# Autodesk Inventor assembly: Chessboard Design
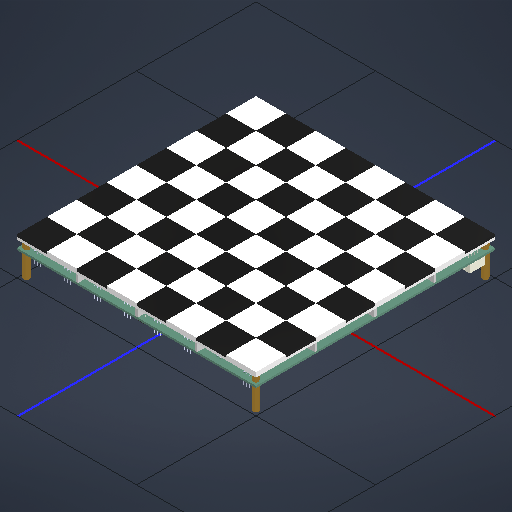
[picture p0: Inventor's stored thumbnail of the model, 512x512]
Saved by Autodesk Inventor 2026 (Build 300175000, 175)
## iProperties
Created: 2025-04-19
Part Number: Chessboard Design
Document SubType Name: Assembly
Designer: ckyiu
Author: ckyiu
## Documents named in this file (6)
- C:\Users\ckyiu\Documents\Projects\Chessboard-Design\Chessboard Design.iam
- C:\Users\ckyiu\Documents\Projects\Chessboard-Design\Assemblies\Chessboard Top.iam
- C:\Users\ckyiu\Documents\Projects\Chessboard-Design\Assemblies\PCBs\Chessboard Hardware Model.iam
- C:\Users\ckyiu\Documents\Projects\Chessboard-Design\Parts\Square Holder Support.ipt
- C:\Users\ckyiu\Documents\Projects\Chessboard-Design\Parts\Standoffs\M2.5 F-F Standoff 6mm.ipt
- C:\Users\ckyiu\Documents\Projects\Chessboard-Design\Parts\Standoffs\M2.5 F-M Standoff 20mm.ipt
## Components (11 placed, 5 different names)
1. Chessboard Top:1 [sub-assembly] — Flush:1, Flush:2, Mate:2
2. Chessboard Hardware Model:1 [sub-assembly] — Flush:1, Flush:2, Flush:3, Flush:4, Mate:1, Insert:1, Angle:1, Insert:2, Angle:2, Insert:3, Angle:3, Insert:4, Angle:4, Insert:5, Insert:6, Insert:7, Insert:8
3. Square Holder Support:1 — Flush:3, Flush:4, Mate:1, Mate:2
4. M2.5 F-F Standoff 6mm:1 — Insert:1, Angle:1, Angle:5
5. M2.5 F-F Standoff 6mm:2 — Insert:4, Angle:4, Angle:7
6. M2.5 F-F Standoff 6mm:3 — Insert:3, Angle:3, Angle:6
7. M2.5 F-F Standoff 6mm:4 — Insert:2, Angle:2, Angle:8
8. M2.5 F-M Standoff 20mm:1 — Insert:5, Angle:5
9. M2.5 F-M Standoff 20mm:2 — Insert:6, Angle:8
10. M2.5 F-M Standoff 20mm:3 — Insert:7, Angle:6
11. M2.5 F-M Standoff 20mm:4 — Insert:8, Angle:7
## Relationships (22: Insert 8, Angle 8, Flush 4, Mate 2)
- Flush:1: Chessboard Top:1 ↔ Chessboard Hardware Model:1
- Flush:2: Chessboard Top:1 ↔ Chessboard Hardware Model:1
- Flush:3: Chessboard Hardware Model:1 ↔ Square Holder Support:1
- Flush:4: Chessboard Hardware Model:1 ↔ Square Holder Support:1
- Mate:1: Chessboard Hardware Model:1 ↔ Square Holder Support:1
- Mate:2: Chessboard Top:1 ↔ Square Holder Support:1
- Insert:1: Chessboard Hardware Model:1 ↔ M2.5 F-F Standoff 6mm:1
- Angle:1 (0 deg): Chessboard Hardware Model:1 ↔ M2.5 F-F Standoff 6mm:1
- Insert:2: Chessboard Hardware Model:1 ↔ M2.5 F-F Standoff 6mm:4
- Angle:2 (0 deg): Chessboard Hardware Model:1 ↔ M2.5 F-F Standoff 6mm:4
- Insert:3: Chessboard Hardware Model:1 ↔ M2.5 F-F Standoff 6mm:3
- Angle:3 (0 deg): Chessboard Hardware Model:1 ↔ M2.5 F-F Standoff 6mm:3
- Insert:4: Chessboard Hardware Model:1 ↔ M2.5 F-F Standoff 6mm:2
- Angle:4 (0 deg): Chessboard Hardware Model:1 ↔ M2.5 F-F Standoff 6mm:2
- Insert:5: Chessboard Hardware Model:1 ↔ M2.5 F-M Standoff 20mm:1
- Insert:6: Chessboard Hardware Model:1 ↔ M2.5 F-M Standoff 20mm:2
- Insert:7: Chessboard Hardware Model:1 ↔ M2.5 F-M Standoff 20mm:3
- Insert:8: Chessboard Hardware Model:1 ↔ M2.5 F-M Standoff 20mm:4
- Angle:5 (0 deg): M2.5 F-F Standoff 6mm:1 ↔ M2.5 F-M Standoff 20mm:1
- Angle:6 (0 deg): M2.5 F-F Standoff 6mm:3 ↔ M2.5 F-M Standoff 20mm:3
- Angle:7 (0 deg): M2.5 F-F Standoff 6mm:2 ↔ M2.5 F-M Standoff 20mm:4
- Angle:8 (0 deg): M2.5 F-F Standoff 6mm:4 ↔ M2.5 F-M Standoff 20mm:2
